# Autodesk Inventor assembly: Coupler lift long left bracket + pulleys
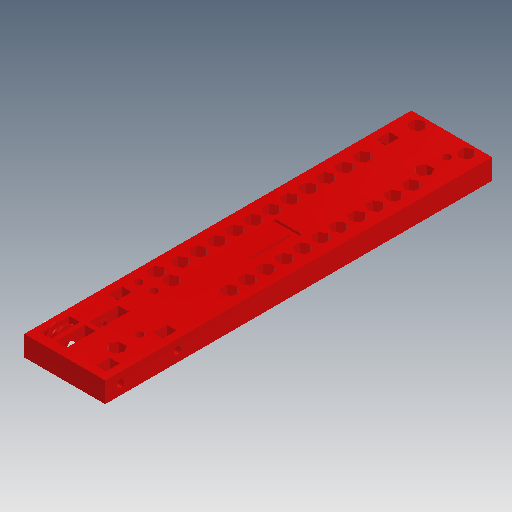
[picture p0: Inventor's stored thumbnail of the model, 512x512]
Saved by Autodesk Inventor 2020 (Build 240168000, 168)
## iProperties
Created: 2019-12-12
Part Number: Coupler lift long left bracket + pulleys
Document SubType Name: Assembly
Designer: ball
Author: ball
## Documents named in this file (4)
- C:\FTC\FTC8863CAD\2019 Robot\Delivery\Coupler lift long left bracket + pulleys.iam
- C:\FTC\FTC8863CAD\2019 Robot\Delivery\plastic pulley deep u.ipt
- C:\FTC\FTC8863CAD\StepLibraries\Screws\M3 x 20 HEX HEAD CAP SCREW.ipt
- C:\FTC\FTC8863CAD\2019 Robot\Delivery\Coupler lift long left bracket.ipt
## Components (3 placed, 3 different names)
1. Coupler lift long left bracket:1 — Mate:1, Mate:2, Mate:3, Mate:4
2. plastic pulley deep u:1 — Mate:1, Mate:2
3. M3 x 20 HEX HEAD CAP SCREW:1 — Mate:3, Mate:4
## Relationships (4: Mate 4)
- Mate:1: Coupler lift long left bracket:1 ↔ plastic pulley deep u:1
- Mate:2: Coupler lift long left bracket:1 ↔ plastic pulley deep u:1
- Mate:3: Coupler lift long left bracket:1 ↔ M3 x 20 HEX HEAD CAP SCREW:1
- Mate:4: Coupler lift long left bracket:1 ↔ M3 x 20 HEX HEAD CAP SCREW:1
